# Autodesk Inventor assembly: booth
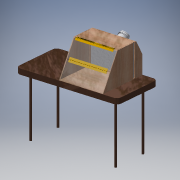
[picture p0: Inventor's stored thumbnail of the model, 180x180]
Saved by Autodesk Inventor 2017 (Build 210142000, 142)
## iProperties
Created: 2019-04-11
Part Number: booth
Document SubType Name: Assembly
Designer: Brian
Author: Brian
## Documents named in this file (20)
- B:\Miniatures\spray booth\compact 14x20 version\booth.iam
- B:\Miniatures\spray booth\compact 14x20 version\Back Side.ipt
- B:\Miniatures\spray booth\compact 14x20 version\Cap Side.ipt
- B:\Miniatures\spray booth\compact 14x20 version\Top Side.ipt
- B:\Miniatures\spray booth\compact 14x20 version\Left Side.ipt
- B:\Miniatures\spray booth\compact 14x20 version\Bottom Base.ipt
- B:\Miniatures\spray booth\compact 14x20 version\Right Side - Rear.ipt
- B:\Miniatures\spray booth\compact 14x20 version\Right Side - Forward.ipt
- B:\Miniatures\spray booth\compact 14x20 version\Filter.ipt
- B:\Miniatures\spray booth\compact 14x20 version\Acrylic Panel - Top.ipt
- B:\Miniatures\spray booth\compact 14x20 version\Acrylic Panel - Bottom.ipt
- B:\Miniatures\spray booth\compact 14x20 version\PianoHingePlate.ipt
- B:\Miniatures\spray booth\compact 14x20 version\dayton1TDT2 $167.ipt
- B:\Miniatures\spray booth\compact 14x20 version\table.ipt
- B:\Miniatures\spray booth\compact 14x20 version\attwood 4000.iam
- B:\Miniatures\spray booth\compact 14x20 version\booth.ipt
- B:\Miniatures\spray booth\compact 14x20 version\Frame - Horizontal.ipt
- B:\Miniatures\spray booth\compact 14x20 version\Frame - Vertical.ipt
- B:\Miniatures\spray booth\textures\Wrinkled Paper.jpg
- B:\Miniatures\spray booth\textures\images.png
## Components (19 placed, 16 different names)
1. Back Side:1
2. Cap Side:1 — Rigid:2
3. Top Side:1 — Mate:2
4. Left Side:1
5. Bottom Base:1 — Slider:2, Rigid:1
6. Right Side - Rear:1
7. Right Side - Forward:1 — Mate:4, Mate:9
8. Filter:1 — Slider:3
9. Acrylic Panel - Top:1 — Flush:1, Mate:7, Flush:9, Mate:10, Flush:2, Mate:11
10. Acrylic Panel - Bottom:1 — Mate:12, Flush:3, Mate:13
11. PianoHingePlate:1 — Flush:1, Mate:7, Flush:9, Rotational:1
12. PianoHingePlate:2 — Mate:2, Mate:4, Rotational:1, Mate:9
13. PianoHingePlate:3 — Mate:10, Flush:2, Mate:11, Rotational:2
14. PianoHingePlate:4 — Rotational:2, Mate:12, Flush:3, Mate:13
15. dayton1TDT2 $167:2 — Rigid:1
16. attwood 4000:1 [sub-assembly] — Rigid:2
17. table:1 — Slider:2
18. Frame - Horizontal — Slider:3
19. Frame - Vertical
## Component patterns: Filter Frame - Horizontal (1 elements), Filter Frame - Vertical (1 elements)
## Relationships (18: Mate 8, Flush 4, RevoluteJoint 2, TranslationJoint 2, WeldJoint 2)
- Mate:2: Top Side:1 ↔ PianoHingePlate:2
- Mate:4 (38.1 mm): Right Side - Forward:1 ↔ PianoHingePlate:2
- Flush:1 (38.1 mm): Acrylic Panel - Top:1 ↔ PianoHingePlate:1
- Mate:7: Acrylic Panel - Top:1 ↔ PianoHingePlate:1
- Flush:9 (-1.27 mm): Acrylic Panel - Top:1 ↔ PianoHingePlate:1
- Rotational:1 [RevoluteJoint]: PianoHingePlate:1 ↔ PianoHingePlate:2
- Mate:9 (6.35 mm): Right Side - Forward:1 ↔ PianoHingePlate:2
- Mate:10: Acrylic Panel - Top:1 ↔ PianoHingePlate:3
- Flush:2 (38.1 mm): Acrylic Panel - Top:1 ↔ PianoHingePlate:3
- Mate:11: Acrylic Panel - Top:1 ↔ PianoHingePlate:3
- Rotational:2 [RevoluteJoint]: PianoHingePlate:3 ↔ PianoHingePlate:4
- Mate:12: Acrylic Panel - Bottom:1 ↔ PianoHingePlate:4
- Flush:3 (38.1 mm): Acrylic Panel - Bottom:1 ↔ PianoHingePlate:4
- Mate:13: Acrylic Panel - Bottom:1 ↔ PianoHingePlate:4
- Slider:2 [TranslationJoint]: Bottom Base:1 ↔ table:1
- Rigid:1 [WeldJoint]: Bottom Base:1 ↔ dayton1TDT2 $167:2
- Rigid:2 [WeldJoint]: Cap Side:1 ↔ attwood 4000:1
- Slider:3 [TranslationJoint]: Filter:1 ↔ Frame - Horizontal
## Named parameters: filter_width = 508 mm, filter_frame = 12.7 mm, base_depth = 584.2 mm, plywood_thickness = 8.73125 mm, twobytwo_height = 38.1 mm, dowel_thickness = 12.7 mm, plenum_depth = 101.6 mm, filter_thickness = 25.4 mm, filter_height = 355.6 mm, acrylic_thickness = 6.35 mm
